# Autodesk Inventor assembly: 3.25" Traction Wheel, Square Insert
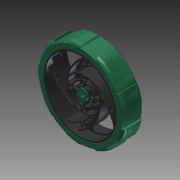
[picture p0: Inventor's stored thumbnail of the model, 180x180]
Saved by Autodesk Inventor 2016 (Build 200138000, 138)
## iProperties
Company: Bots 'n' Stuff
Created: 2014-08-29
Document SubType Name: Assembly
Designer: Jordan Kiesel
Vendor: VEX Robotics, Inc.
Mass: 54.4672 g
Surface Area: 417.393 cm^2
Volume: 47.139 cm^3
Density: 1.15546 g/cm^3
Author: Jordan Kiesel
Title: 3.25" Traction Wheel, Square Insert
## Documents named in this file (3)
- C:\Users\Jordan\Documents\Robotics\CAD\2015 BNS CAD Library (beta)\Motion\Wheels & Rollers\3.25'' Traction Wheel, Free Spinning Insert.iam
- C:\Users\Jordan\Documents\Robotics\CAD\2015 BNS CAD Library (beta)\Motion\Wheels & Rollers\Reference Parts\3.25'' Traction Wheels\3.25'' Traction Wheel.iam
- C:\Users\Jordan\Documents\Robotics\CAD\2015 BNS CAD Library (beta)\Motion\Reference Parts\Free Spinning Gear Insert.ipt
## Components (3 placed, 2 different names)
1. 3.25'' Traction Wheel:1 [sub-assembly] — Mate:3, Mate:6
2. Free Spinning Gear Insert:1 — Mate:3
3. Free Spinning Gear Insert:2 — Mate:6
## Relationships (6: Mate 6)
- [Mate] (0.0254 mm): 3.25'' Traction Wheel:1 ↔ Free Spinning Gear Insert:1
- [Mate] (0.0254 mm): 3.25'' Traction Wheel:1 ↔ Free Spinning Gear Insert:1
- Mate:3: 3.25'' Traction Wheel:1 ↔ Free Spinning Gear Insert:1
- [Mate] (0.0254 mm): 3.25'' Traction Wheel:1 ↔ Free Spinning Gear Insert:2
- [Mate] (0.0254 mm): 3.25'' Traction Wheel:1 ↔ Free Spinning Gear Insert:2
- Mate:6: 3.25'' Traction Wheel:1 ↔ Free Spinning Gear Insert:2
